# Autodesk Inventor assembly: Drive Block
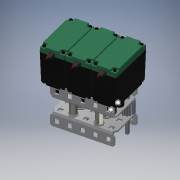
[picture p0: Inventor's stored thumbnail of the model, 180x180]
Saved by Autodesk Inventor 2017 (Build 210142000, 142)
## iProperties
Created: 2017-07-31
Part Number: Drive Block
Document SubType Name: Assembly
Designer: ollyb
Author: ollyb
## Documents named in this file (7)
- C:\Users\ollyb\OneDrive\Documents\Vex Parts\Stuff i am working on\Drive Block.iam
- C:\Users\ollyb\OneDrive\Documents\Vex Parts\Metal\C-Channels\Assembly4.iam
- C:\Users\ollyb\OneDrive\Documents\Vex Parts\Motors & Sensors\2-Wire Motor 393.iam
- C:\Users\ollyb\OneDrive\Documents\Vex Parts\Standoffs & Couplers\Standoff 0.50''.ipt
- C:\Users\ollyb\OneDrive\Documents\Vex Parts\Washers & Spacers\Washer, Steel, 0.032''.ipt
- C:\Users\ollyb\OneDrive\Documents\Vex Parts\Drive Shafts\Drive Shaft 2''.ipt
- C:\Users\ollyb\OneDrive\Documents\Vex Parts\Spur Gears\High Strength 12-tooth Gear.ipt
## Components (37 placed, 6 different names)
1. Assembly4:1 [sub-assembly] — Mate:1, Mate:2, Mate:3, Mate:4, Mate:5, Mate:6, Mate:7, Mate:8, Mate:9, Mate:10, Mate:11, Mate:12, Mate:13, Mate:14, Mate:15, Mate:16, Mate:17, Insert:2, Insert:4, Insert:5, Mate:35, Mate:36, Mate:37, Mate:38, Mate:39, Mate:40, Mate:41, Mate:42, Mate:43, Mate:44, Mate:64, Mate:69, Mate:70, Mate:71, Mate:72, Mate:74, Mate:75
2. 2-Wire Motor 393:1 [sub-assembly] — Mate:1, Mate:2, Mate:3, Insert:1
3. 2-Wire Motor 393:2 [sub-assembly] — Mate:4, Mate:5, Mate:6
4. 2-Wire Motor 393:3 [sub-assembly] — Mate:7, Mate:8, Mate:9, Insert:3
5. Standoff 0.50'':1 — Mate:20, Mate:21, Mate:26, Mate:28, Mate:29, Mate:30
6. Standoff 0.50'':2 — Mate:24, Mate:25, Mate:31, Mate:32
7. Standoff 0.50'':3 — Mate:18, Mate:19, Mate:33, Mate:34
8. Standoff 0.50'':4 — Mate:22, Mate:23, Mate:27
9. Washer, Steel, 0.032'':1 — Mate:12, Mate:13, Mate:22, Mate:23
10. Washer, Steel, 0.032'':2 — Mate:14, Mate:15, Mate:18, Mate:19
11. Washer, Steel, 0.032'':3 — Mate:16, Mate:17, Mate:24, Mate:25
12. Washer, Steel, 0.032'':4 — Mate:27, Mate:28
13. Washer, Steel, 0.032'':5 — Mate:31, Mate:32
14. Washer, Steel, 0.032'':6 — Mate:26, Mate:29, Mate:30
15. Washer, Steel, 0.032'':7 — Mate:33, Mate:34
16. Washer, Steel, 0.032'':8 — Mate:10, Mate:11, Mate:20, Mate:21
17. Assembly4:2 [sub-assembly] — Mate:73, Mate:74, Mate:75
18. Drive Shaft 2'':1 — Insert:2, Mate:54, Mate:55
19. Drive Shaft 2'':2 — Insert:3, Mate:57, Mate:58
20. Drive Shaft 2'':3 — Insert:1, Mate:48, Mate:49
21. High Strength 12-tooth Gear:1 — Mate:48, Mate:49, Mate:50, Rotation:4, Mate:68
22. High Strength 12-tooth Gear:2 — Mate:54, Mate:55, Mate:56, Rotation:2, Rotation:3, Mate:66
23. High Strength 12-tooth Gear:3 — Mate:45, Mate:46, Mate:47, Mate:57, Mate:58, Mate:59, Rotation:1, Mate:63
24. High Strength 12-tooth Gear:4 — Mate:51, Mate:52, Mate:53, Rotation:3, Rotation:4, Mate:67
25. Drive Shaft 2'':4 — Insert:4, Mate:51, Mate:52
26. Drive Shaft 2'':5 — Insert:5, Mate:60, Mate:61
27. Washer, Steel, 0.032'':9 — Mate:37, Mate:38, Mate:53
28. Washer, Steel, 0.032'':10 — Mate:39, Mate:40, Mate:56
29. Washer, Steel, 0.032'':11 — Mate:41, Mate:42, Mate:62
30. Washer, Steel, 0.032'':12 — Mate:43, Mate:44, Mate:59
31. Washer, Steel, 0.032'':13 — Mate:68, Mate:69, Mate:73
32. Washer, Steel, 0.032'':14 — Mate:35, Mate:36, Mate:50
33. Washer, Steel, 0.032'':15 — Mate:63, Mate:64
34. Washer, Steel, 0.032'':16 — Mate:65, Mate:72
35. Washer, Steel, 0.032'':17 — Mate:66, Mate:71
36. Washer, Steel, 0.032'':18 — Mate:67, Mate:70
37. High Strength 12-tooth Gear:5 — Mate:60, Mate:61, Mate:62, Rotation:1, Rotation:2, Mate:65
## Relationships (84: Mate 75, Insert 5, RelateRotation 4)
- Mate:1: Assembly4:1 ↔ 2-Wire Motor 393:1
- Mate:2: Assembly4:1 ↔ 2-Wire Motor 393:1
- Mate:3: Assembly4:1 ↔ 2-Wire Motor 393:1
- Mate:4: Assembly4:1 ↔ 2-Wire Motor 393:2
- Mate:5: Assembly4:1 ↔ 2-Wire Motor 393:2
- Mate:6: Assembly4:1 ↔ 2-Wire Motor 393:2
- Mate:7: Assembly4:1 ↔ 2-Wire Motor 393:3
- Mate:8: Assembly4:1 ↔ 2-Wire Motor 393:3
- Mate:9: Assembly4:1 ↔ 2-Wire Motor 393:3
- Mate:10: Assembly4:1 ↔ Washer, Steel, 0.032'':8
- Mate:11: Assembly4:1 ↔ Washer, Steel, 0.032'':8
- Mate:12: Assembly4:1 ↔ Washer, Steel, 0.032'':1
- Mate:13: Assembly4:1 ↔ Washer, Steel, 0.032'':1
- Mate:14: Assembly4:1 ↔ Washer, Steel, 0.032'':2
- Mate:15: Assembly4:1 ↔ Washer, Steel, 0.032'':2
- Mate:16: Assembly4:1 ↔ Washer, Steel, 0.032'':3
- Mate:17: Assembly4:1 ↔ Washer, Steel, 0.032'':3
- Mate:18: Standoff 0.50'':3 ↔ Washer, Steel, 0.032'':2
- Mate:19: Standoff 0.50'':3 ↔ Washer, Steel, 0.032'':2
- Mate:20: Standoff 0.50'':1 ↔ Washer, Steel, 0.032'':8
- Mate:21: Standoff 0.50'':1 ↔ Washer, Steel, 0.032'':8
- Mate:22: Standoff 0.50'':4 ↔ Washer, Steel, 0.032'':1
- Mate:23: Standoff 0.50'':4 ↔ Washer, Steel, 0.032'':1
- Mate:24: Standoff 0.50'':2 ↔ Washer, Steel, 0.032'':3
- Mate:25: Standoff 0.50'':2 ↔ Washer, Steel, 0.032'':3
- Mate:26: Standoff 0.50'':1 ↔ Washer, Steel, 0.032'':6
- Mate:27: Standoff 0.50'':4 ↔ Washer, Steel, 0.032'':4
- Mate:28: Standoff 0.50'':1 ↔ Washer, Steel, 0.032'':4
- Mate:29: Standoff 0.50'':1 ↔ Washer, Steel, 0.032'':6
- Mate:30: Standoff 0.50'':1 ↔ Washer, Steel, 0.032'':6
- Mate:31: Standoff 0.50'':2 ↔ Washer, Steel, 0.032'':5
- Mate:32: Standoff 0.50'':2 ↔ Washer, Steel, 0.032'':5
- Mate:33: Standoff 0.50'':3 ↔ Washer, Steel, 0.032'':7
- Mate:34: Standoff 0.50'':3 ↔ Washer, Steel, 0.032'':7
- Insert:1: 2-Wire Motor 393:1 ↔ Drive Shaft 2'':3
- Insert:2 (-15.24 mm): Assembly4:1 ↔ Drive Shaft 2'':1
- Insert:3: 2-Wire Motor 393:3 ↔ Drive Shaft 2'':2
- Insert:4 (-15.24 mm): Assembly4:1 ↔ Drive Shaft 2'':4
- Insert:5 (-15.24 mm): Assembly4:1 ↔ Drive Shaft 2'':5
- Mate:35: Assembly4:1 ↔ Washer, Steel, 0.032'':14
- Mate:36: Assembly4:1 ↔ Washer, Steel, 0.032'':14
- Mate:37: Assembly4:1 ↔ Washer, Steel, 0.032'':9
- Mate:38: Assembly4:1 ↔ Washer, Steel, 0.032'':9
- Mate:39: Assembly4:1 ↔ Washer, Steel, 0.032'':10
- Mate:40: Assembly4:1 ↔ Washer, Steel, 0.032'':10
- Mate:41: Assembly4:1 ↔ Washer, Steel, 0.032'':11
- Mate:42: Assembly4:1 ↔ Washer, Steel, 0.032'':11
- Mate:43: Assembly4:1 ↔ Washer, Steel, 0.032'':12
- Mate:44: Assembly4:1 ↔ Washer, Steel, 0.032'':12
- Mate:45: High Strength 12-tooth Gear:3
- Mate:46: High Strength 12-tooth Gear:3
- Mate:47: High Strength 12-tooth Gear:3
- Mate:48: Drive Shaft 2'':3 ↔ High Strength 12-tooth Gear:1
- Mate:49: Drive Shaft 2'':3 ↔ High Strength 12-tooth Gear:1
- Mate:50: High Strength 12-tooth Gear:1 ↔ Washer, Steel, 0.032'':14
- Mate:51: High Strength 12-tooth Gear:4 ↔ Drive Shaft 2'':4
- Mate:52: High Strength 12-tooth Gear:4 ↔ Drive Shaft 2'':4
- Mate:53: High Strength 12-tooth Gear:4 ↔ Washer, Steel, 0.032'':9
- Mate:54: Drive Shaft 2'':1 ↔ High Strength 12-tooth Gear:2
- Mate:55: Drive Shaft 2'':1 ↔ High Strength 12-tooth Gear:2
- Mate:56: High Strength 12-tooth Gear:2 ↔ Washer, Steel, 0.032'':10
- Mate:57: Drive Shaft 2'':2 ↔ High Strength 12-tooth Gear:3
- Mate:58: Drive Shaft 2'':2 ↔ High Strength 12-tooth Gear:3
- Mate:59: High Strength 12-tooth Gear:3 ↔ Washer, Steel, 0.032'':12
- Mate:60: Drive Shaft 2'':5 ↔ High Strength 12-tooth Gear:5
- Mate:61: Drive Shaft 2'':5 ↔ High Strength 12-tooth Gear:5
- Mate:62: Washer, Steel, 0.032'':11 ↔ High Strength 12-tooth Gear:5
- Rotation:1 [RelateRotation] (1 ul): High Strength 12-tooth Gear:3 ↔ High Strength 12-tooth Gear:5
- Rotation:2 [RelateRotation] (1 ul): High Strength 12-tooth Gear:2 ↔ High Strength 12-tooth Gear:5
- Rotation:3 [RelateRotation] (1 ul): High Strength 12-tooth Gear:2 ↔ High Strength 12-tooth Gear:4
- Rotation:4 [RelateRotation] (1 ul): High Strength 12-tooth Gear:1 ↔ High Strength 12-tooth Gear:4
- Mate:63: High Strength 12-tooth Gear:3 ↔ Washer, Steel, 0.032'':15
- Mate:64: Assembly4:1 ↔ Washer, Steel, 0.032'':15
- Mate:65: Washer, Steel, 0.032'':16 ↔ High Strength 12-tooth Gear:5
- Mate:66: High Strength 12-tooth Gear:2 ↔ Washer, Steel, 0.032'':17
- Mate:67: High Strength 12-tooth Gear:4 ↔ Washer, Steel, 0.032'':18
- Mate:68: High Strength 12-tooth Gear:1 ↔ Washer, Steel, 0.032'':13
- Mate:69: Assembly4:1 ↔ Washer, Steel, 0.032'':13
- Mate:70: Assembly4:1 ↔ Washer, Steel, 0.032'':18
- Mate:71: Assembly4:1 ↔ Washer, Steel, 0.032'':17
- Mate:72: Assembly4:1 ↔ Washer, Steel, 0.032'':16
- Mate:73: Assembly4:2 ↔ Washer, Steel, 0.032'':13
- Mate:74: Assembly4:1 ↔ Assembly4:2
- Mate:75: Assembly4:1 ↔ Assembly4:2
